# Autodesk Inventor assembly: FullGripperBlock
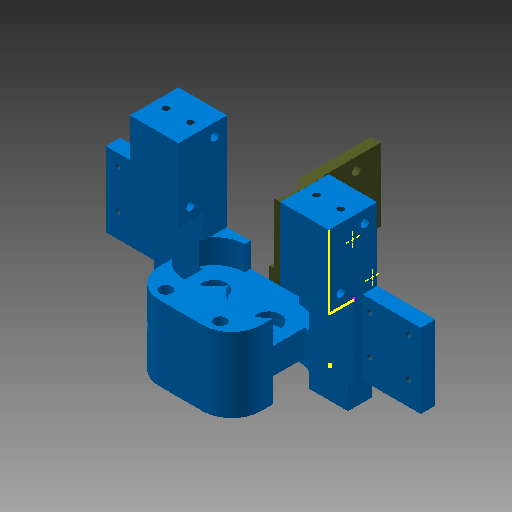
[picture p0: Inventor's stored thumbnail of the model, 512x512]
Saved by Autodesk Inventor 2019 (Build 230136000, 136)
## iProperties
Created: 2019-10-11
Part Number: FullGripperBlock
Document SubType Name: Assembly
Designer: james
Author: james
## Documents named in this file (3)
- F:\JimsDesign\Jims2020FTC\FullGripperBlock.iam
- F:\JimsDesign\Jims2020FTC\BottomOfGripperBlock.ipt
- F:\JimsDesign\Jims2020FTC\MiddleOfGripperWithPlate.iam
## Components (2 placed, 2 different names)
1. MiddleOfGripperWithPlate:1 [sub-assembly] — Mate:1, Mate:2, Mate:3
2. BottomOfGripperBlock:1 — Mate:1, Mate:2, Mate:3
## Relationships (3: Mate 3)
- Mate:1: MiddleOfGripperWithPlate:1 ↔ BottomOfGripperBlock:1
- Mate:2: MiddleOfGripperWithPlate:1 ↔ BottomOfGripperBlock:1
- Mate:3: MiddleOfGripperWithPlate:1 ↔ BottomOfGripperBlock:1
